# Autodesk Inventor assembly: 536288 ADN-40-100-I-P-A---(0)
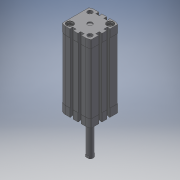
[picture p0: Inventor's stored thumbnail of the model, 180x180]
Saved by Autodesk Inventor 2018 (Build 220112000, 112)
## iProperties
Category: PARTsolutions
Company: FESTO
Part Number: 536288 ADN-40-100-I-P-A---(0)
Catalog Web Link: www.cadenas.de
Description: ADN (mp)-Compact cylinder, Modular system
Vendor: FESTO
Document SubType Name: Assembly
Designer: partserver
Manufacturer: FESTO
Mass: 716 g
Surface Area: 857.246 cm^2
Volume: 258.859 cm^3
Density: 2.76598 g/cm^3
PSOL_IDENT_0: {ATYP=ASSISTANT},{DATA=script=$CADENAS_DATA/23d-libs/festo/webfesto.vbb/&M_FAMILY=ADN&M_GROUP=01&M_P
PSOL_IDENT_1: ARTNO=536288&IDCODE1=ADN-40-100-I-P-A&IDCODE2=&C_ADN_AF=A&C_ADN_DA=P&C_ADN_DM=40&C_ADN_GA=I&C_ADN_HE
PSOL_IDENT_2: AD=ADN&HUB=100&VCSD_UPDATE_YYIDENT11=ADN-40-100-I-P-A&customer_number_cns=&MATES=1&LOD=HI&LOCKERP=1}
NB: 536288 ADN-40-100-I-P-A---(0)
NN: ADN (mp)
NT: Compact cylinder, Modular system
NBSYN: $TNR. $TYP.-$HUB.-$TH.-$DF.-$GA.$QN.$S2S20N.$K2N.$K5N.$K8N.$K10N.$S6N.$S10N.$S11N.$R3N.$S1N.$TLN.$TTN.$R8N.$EX4N.$TXTN.---($HUBST.)
LINA: 536288 ADN-40-100-I-P-A---(0)
CATALOG: Festo
OFFICIAL_STANDARD_NUMBERS: ISO 21287
TNR: 536288
TYP: ADN-40
KDM: 40
HUB: 100
TH: I
HUBST: 0
DF: P
GA: A
Q: -
S2S20: -
K2: 0
K5: -
K8: 0
K10: -
S6: -
S10: -
S11: -
R3: -
S1: -
TL: -
TT: -
R8: -
ATEX: -
TXT: -
A: 19
A1: 22
AF: 16
AF1: 20
AF2: 0
AF3: 14
AF5: 14
AF7: 16
B: 35
B1: 27
BG: 26
BG1: 26
DA: 9
D1: 9
D2: 17
D3: 8
D4: M5
D5: 33
D20: 4.5
D21: 8
E: 54.5
EE: G1/8
EE1: M5
FB: 5
G: 15
J: 15
KF: M8
KF1: M10
KF2: -
KF3: M6
KF5: M6
KF7: M8
KK: M10x1.25
KK1: M12x1.25
LA: 5
LA1: 5
MM: 12
MM1: 16
PL: 8.2
RR: 5.1
RT: M6
SF: 10
SF1: 13
SF3: 10
TG: 38
U1: 8
U2: 15
VD: 9.5
VD1: 6.4
WH: 6.1
WH0: 6.1
WH1: 18
WH2: 12.5
WH3: 6.6
WL: 4.7
WL1: 6.5
W1: 2.1
W2: 61
W3: 10
W4: 6
W20: 3.3
W21: 4.7
W22: 3
W23: 2.6
W25: 2.6
W27: 3.3
Y1: 0.4
Y2: 0.6
ZA: 45
ZB: 51.1
ZB1: 62.9
ZB2: 51.7
ZB6: 57.5
ZM: 58.6
ZM2: 59.7
CNSMASSEXACT: 0.716
SUPPLIER: FESTO
ARTICLENO: 536288 ADN-40-100-I-P-A---(0)
BOMINFO: 536288 ADN-40-100-I-P-A---(0)
CREATOR: CADENAS GmbH
Title: 536288 ADN-40-100-I-P-A---(0)
Author: Cadenas PARTsolutions
Comments: Compact cylinder, Modular system
## Documents named in this file (3)
- C:\Users\Francesco\no-brim\Meccanica\Progetto Inventor no-brim\Parti\Pistone salita lama d 40 c 100\AIS2017\536288 ADN-40-100-I-P-A---(0).iam
- C:\Users\Francesco\no-brim\Meccanica\Progetto Inventor no-brim\Parti\Pistone salita lama d 40 c 100\AIS2017\536288 ADN-100-P---(Z).ipt
- C:\Users\Francesco\no-brim\Meccanica\Progetto Inventor no-brim\Parti\Pistone salita lama d 40 c 100\AIS2017\536288 ADN-100-P-I_(KS).ipt
## Components (2 placed, 2 different names)
1. 536288 ADN-100-P---(Z):1 — CYLINDER_XY@1 <-> PISTON_XY@2, CYLINDER_Z@1 <-> PISTON_Z@2, CYLINDER_YZ@1 <-> PISTON_YZ@2
2. 536288 ADN-100-P-I_(KS):1 — CYLINDER_XY@1 <-> PISTON_XY@2, CYLINDER_Z@1 <-> PISTON_Z@2, CYLINDER_YZ@1 <-> PISTON_YZ@2
## Relationships (3: Mate 2, Angle 1)
- CYLINDER_XY@1 <-> PISTON_XY@2 [Mate]: 536288 ADN-100-P---(Z):1 ↔ 536288 ADN-100-P-I_(KS):1
- CYLINDER_Z@1 <-> PISTON_Z@2 [Mate]: 536288 ADN-100-P---(Z):1 ↔ 536288 ADN-100-P-I_(KS):1
- CYLINDER_YZ@1 <-> PISTON_YZ@2 [Angle] (0 deg): 536288 ADN-100-P---(Z):1 ↔ 536288 ADN-100-P-I_(KS):1
